# Autodesk Inventor assembly: Actuador electrico
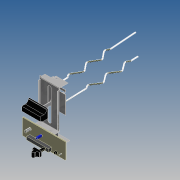
[picture p0: Inventor's stored thumbnail of the model, 180x180]
Saved by Autodesk Inventor 2016 (Build 200138000, 138)
## iProperties
Created: 2016-05-25
Part Number: Actuador electrico
Document SubType Name: Assembly
Designer: Familia
Author: Familia
## Documents named in this file (9)
- C:\Users\Familia\Desktop\Tostadora\Ensambles\Actuador electrico.iam
- C:\Users\Familia\Desktop\Tostadora\Partes\Targeta electrica.ipt
- C:\Users\Familia\Desktop\Tostadora\Partes\Soporte 1.ipt
- C:\Users\Familia\Desktop\Tostadora\Partes\Porta actuador.ipt
- C:\Users\Familia\Desktop\Tostadora\Partes\Eje guia.ipt
- C:\Users\Familia\Desktop\Tostadora\Partes\Barra expulsora 1.ipt
- C:\Users\Familia\Desktop\Tostadora\Partes\Barra expulsora 2.ipt
- C:\Users\Familia\Desktop\Tostadora\Partes\Boton de extraccion.ipt
- C:\Users\Familia\Desktop\Tostadora\Partes\Boton de temperaturas.ipt
## Components (8 placed, 8 different names)
1. Targeta electrica:1 — Flush:1, Flush:2, Flush:3, Mate:1, Flush:4, Mate:2, Mate:3, Mate:11, Mate:12
2. Soporte 1:1 — Mate:1, Flush:4, Mate:2, Flush:5, Mate:4, Mate:5, Mate:6
3. Porta actuador:1 — Mate:3, Flush:5, Mate:4, Mate:7, Flush:6, Mate:8, Flush:7, Mate:9, Mate:10
4. Eje guia:1 — Mate:5, Mate:6
5. Barra expulsora 1:1 — Mate:7, Flush:6
6. Barra expulsora 2:1 — Mate:8, Flush:7
7. Boton de extraccion:1 — Mate:9, Mate:10
8. Boton de temperaturas:1 — Mate:11, Mate:12
## Relationships (19: Mate 12, Flush 7)
- Flush:1: Targeta electrica:1
- Flush:2: Targeta electrica:1
- Flush:3: Targeta electrica:1
- Mate:1: Targeta electrica:1 ↔ Soporte 1:1
- Flush:4: Targeta electrica:1 ↔ Soporte 1:1
- Mate:2: Targeta electrica:1 ↔ Soporte 1:1
- Mate:3: Targeta electrica:1 ↔ Porta actuador:1
- Flush:5: Soporte 1:1 ↔ Porta actuador:1
- Mate:4 (3 mm): Soporte 1:1 ↔ Porta actuador:1
- Mate:5: Soporte 1:1 ↔ Eje guia:1
- Mate:6: Soporte 1:1 ↔ Eje guia:1
- Mate:7: Porta actuador:1 ↔ Barra expulsora 1:1
- Flush:6: Porta actuador:1 ↔ Barra expulsora 1:1
- Mate:8: Porta actuador:1 ↔ Barra expulsora 2:1
- Flush:7: Porta actuador:1 ↔ Barra expulsora 2:1
- Mate:9: Porta actuador:1 ↔ Boton de extraccion:1
- Mate:10: Porta actuador:1 ↔ Boton de extraccion:1
- Mate:11: Targeta electrica:1 ↔ Boton de temperaturas:1
- Mate:12: Targeta electrica:1 ↔ Boton de temperaturas:1
